# Autodesk Inventor assembly: bottom box with container
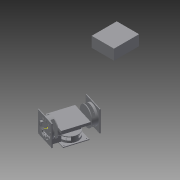
[picture p0: Inventor's stored thumbnail of the model, 180x180]
Saved by Autodesk Inventor 2015 (Build 190159000, 159)
## iProperties
Created: 2014-09-09
Part Number: bottom box with container
Document SubType Name: Assembly
Designer: ericd_000
Author: ericd_000
## Documents named in this file (9)
- C:\Users\ericd_000\Dropbox\GitHub\initial_cad\eric_cad\bottom box with container.iam
- C:\Users\ericd_000\Dropbox\GitHub\initial_cad\eric_cad\brain box bottom.ipt
- C:\Users\ericd_000\Dropbox\GitHub\initial_cad\eric_cad\bbb brick.ipt
- C:\Users\ericd_000\Dropbox\GitHub\initial_cad\eric_cad\anker20Ah.ipt
- C:\Users\ericd_000\Dropbox\GitHub\initial_cad\eric_cad\mini-itx.ipt
- C:\Users\ericd_000\Dropbox\GitHub\initial_cad\eric_cad\dlink5portswitch.ipt
- C:\Users\ericd_000\Dropbox\GitHub\initial_cad\eric_cad\stark24v10ahbattery.ipt
- C:\Users\ericd_000\Dropbox\GitHub\initial_cad\eric_cad\small24v2600mahbattery.ipt
- C:\Users\ericd_000\Dropbox\GitHub\initial_cad\eric_cad\bayonet container 8.ipt
## Components (13 placed, 8 different names)
1. brain box bottom:1 — Mate:1, Mate:2, Mate:11, Mate:13, Mate:16, Mate:17, Mate:18, Mate:21, Mate:25, Mate:26, Mate:27, Mate:29, Mate:30, Mate:32, Mate:33, Mate:34, Mate:35, Mate:36, Mate:37
2. bbb brick:1 — Mate:1, Mate:2
3. anker20Ah:1 — Mate:11, Mate:12
4. anker20Ah:2 — Mate:12, Mate:13
5. mini-itx:1 — Mate:30, Mate:31
6. dlink5portswitch:1 — Mate:28, Mate:29, Mate:31
7. stark24v10ahbattery:1
8. small24v2600mahbattery:1 — Mate:16, Mate:17
9. small24v2600mahbattery:3 — Mate:18, Mate:21
10. small24v2600mahbattery:4
11. bayonet container 8:1 — Mate:25, Mate:26, Mate:27, Mate:28
12. bayonet container 8:2 — Mate:32, Mate:33, Mate:34
13. bayonet container 8:3 — Mate:35, Mate:36, Mate:37
## Relationships (22: Mate 22)
- Mate:1: brain box bottom:1 ↔ bbb brick:1
- Mate:2 (2.54 mm): brain box bottom:1 ↔ bbb brick:1
- Mate:11: brain box bottom:1 ↔ anker20Ah:1
- Mate:12 (2.54 mm): anker20Ah:1 ↔ anker20Ah:2
- Mate:13: brain box bottom:1 ↔ anker20Ah:2
- Mate:16: brain box bottom:1 ↔ small24v2600mahbattery:1
- Mate:17 (0.762 mm): brain box bottom:1 ↔ small24v2600mahbattery:1
- Mate:18: brain box bottom:1 ↔ small24v2600mahbattery:3
- Mate:21: brain box bottom:1 ↔ small24v2600mahbattery:3
- Mate:25: brain box bottom:1 ↔ bayonet container 8:1
- Mate:26: brain box bottom:1 ↔ bayonet container 8:1
- Mate:27: brain box bottom:1 ↔ bayonet container 8:1
- Mate:28 (5.08 mm): dlink5portswitch:1 ↔ bayonet container 8:1
- Mate:29 (63.5 mm): brain box bottom:1 ↔ dlink5portswitch:1
- Mate:30 (20.32 mm): brain box bottom:1 ↔ mini-itx:1
- Mate:31 (10.16 mm): mini-itx:1 ↔ dlink5portswitch:1
- Mate:32: brain box bottom:1 ↔ bayonet container 8:2
- Mate:33: brain box bottom:1 ↔ bayonet container 8:2
- Mate:34: brain box bottom:1 ↔ bayonet container 8:2
- Mate:35: brain box bottom:1 ↔ bayonet container 8:3
- Mate:36: brain box bottom:1 ↔ bayonet container 8:3
- Mate:37: brain box bottom:1 ↔ bayonet container 8:3
